# Autodesk Inventor assembly: UmlenkrolleHalterHeavy
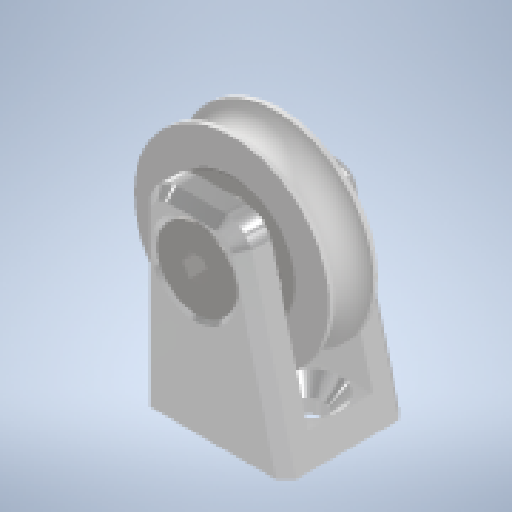
[picture p0: Inventor's stored thumbnail of the model, 512x512]
Saved by Autodesk Inventor 2025 (Build 290162010, 162A)
## iProperties
Created: 2024-11-19
Part Number: UmlenkrolleHalterHeavy
Document SubType Name: Assembly
Designer: Admin
Author: Admin
## Documents named in this file (5)
- C:\Users\Admin\Documents\Inventor\Krandemonstrator\UmlenkrolleHalterHeavy.iam
- C:\Users\Admin\Documents\Inventor\Krandemonstrator\Umlenkrolle.iam
- C:\Users\Admin\Documents\Inventor\Content Center Files\R2025\de-DE\AS 1237 (2.1)\AS 1237 - 4.ipt
- C:\Users\Admin\Documents\Inventor\Content Center Files\R2025\de-DE\DIN 7991(2)\DIN 7991 - M4x12.ipt
- C:\Users\Admin\Documents\Inventor\Krandemonstrator\HalterUmlenkrolleH.ipt
## Components (5 placed, 4 different names)
1. HalterUmlenkrolleH:1 — Starr:3, Passend:1, Starr:1
2. Umlenkrolle:1 [sub-assembly] — Drehbar:1
3. AS 1237 (2.1) 4:1 — Starr:3
4. AS 1237 (2.1) 4:2 — Starr:1, Drehbar:1
5. DIN 7991 M4x12:1 — Passend:1
## Relationships (4: WeldJoint 2, Mate 1, RevoluteJoint 1)
- Starr:3 [WeldJoint]: HalterUmlenkrolleH:1 ↔ AS 1237 (2.1) 4:1
- Passend:1 [Mate]: HalterUmlenkrolleH:1 ↔ DIN 7991 M4x12:1
- Starr:1 [WeldJoint]: HalterUmlenkrolleH:1 ↔ AS 1237 (2.1) 4:2
- Drehbar:1 [RevoluteJoint]: Umlenkrolle:1 ↔ AS 1237 (2.1) 4:2
